# Autodesk Inventor assembly: Wheel Orientation
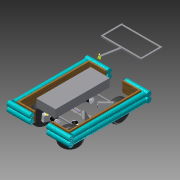
[picture p0: Inventor's stored thumbnail of the model, 180x180]
Saved by Autodesk Inventor 2015 (Build 190159000, 159)
## iProperties
Created: 2016-01-19
Part Number: Wheel Orientation
Document SubType Name: Assembly
Designer: sethbattis
Author: sethbattis
## Documents named in this file (10)
- \\area51\team3566\cad\FRC 2016\Space Claims.iam
- \\area51\team3566\cad\FRC 2016\Wheelbase.ipt
- \\area51\team3566\cad\FRC 2016\Basic Frame.ipt
- \\area51\team3566\cad\FRC 2016\Snow Blower Tire with Gear Box and Mini-CIM.iam
- \\area51\team3566\cad\FRC 2016\Snow Blower Tire with Gear Box and Mini-CIM_MIR.iam
- \\area51\team3566\cad\FRC 2016\Center Truss.ipt
- \\area51\team3566\cad\FRC 2016\Side Bumper.ipt
- \\area51\team3566\cad\FRC 2016\Extension Grappel.ipt
- \\area51\team3566\cad\FRC 2016\Prow rev2.ipt
- \\area51\team3566\cad\FRC 2016\Catapult Base.ipt
## Components (12 placed, 9 different names)
1. Basic Frame:1 — Flush:1, Rigid:1, Rigid:2, Rigid:3, Mate:13, Flush:16, Flush:17, Mate:14, Flush:18, Flush:19, Tangent:1, Mate:19, Mate:20
2. Wheelbase:1 — Flush:1, Rigid:1, Rotational:1, Rotational:2, Rotational:3, Rotational:4, Mate:21
3. Center Truss:1 — Rigid:2, Rigid:3
4. Extension Grappel:1 — Tangent:1
5. Prow rev2:1 — Mate:22
6. Catapult Base:1
7. Side Bumper:2 — Mate:14, Flush:18, Flush:19
8. Side Bumper:1 — Mate:13, Flush:16, Flush:17
9. Snow Blower Tire with Gear Box and Mini-CIM:1 [sub-assembly] — Rotational:1
10. Snow Blower Tire with Gear Box and Mini-CIM:2 [sub-assembly] — Rotational:2
11. Snow Blower Tire with Gear Box and Mini-CIM_MIR:1 [sub-assembly] — Rotational:4
12. Snow Blower Tire with Gear Box and Mini-CIM_MIR:2 [sub-assembly] — Rotational:3
## Relationships (19: Mate 6, Flush 5, RevoluteJoint 4, WeldJoint 3, Tangent 1)
- Flush:1: Basic Frame:1 ↔ Wheelbase:1
- Rigid:1 [WeldJoint]: Basic Frame:1 ↔ Wheelbase:1
- Rotational:1 [RevoluteJoint]: Wheelbase:1 ↔ Snow Blower Tire with Gear Box and Mini-CIM:1
- Rotational:2 [RevoluteJoint]: Wheelbase:1 ↔ Snow Blower Tire with Gear Box and Mini-CIM:2
- Rotational:3 [RevoluteJoint]: Wheelbase:1 ↔ Snow Blower Tire with Gear Box and Mini-CIM_MIR:2
- Rotational:4 [RevoluteJoint]: Wheelbase:1 ↔ Snow Blower Tire with Gear Box and Mini-CIM_MIR:1
- Rigid:2 [WeldJoint]: Basic Frame:1 ↔ Center Truss:1
- Rigid:3 [WeldJoint]: Basic Frame:1 ↔ Center Truss:1
- Mate:13: Basic Frame:1 ↔ Side Bumper:1
- Flush:16: Basic Frame:1 ↔ Side Bumper:1
- Flush:17: Basic Frame:1 ↔ Side Bumper:1
- Mate:14: Basic Frame:1 ↔ Side Bumper:2
- Flush:18: Basic Frame:1 ↔ Side Bumper:2
- Flush:19: Basic Frame:1 ↔ Side Bumper:2
- Tangent:1: Basic Frame:1 ↔ Extension Grappel:1
- Mate:19: Basic Frame:1
- Mate:20: Basic Frame:1
- Mate:21: Wheelbase:1
- Mate:22: Prow rev2:1
